# Autodesk Inventor assembly: Bed
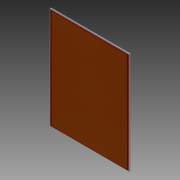
[picture p0: Inventor's stored thumbnail of the model, 180x180]
Saved by Autodesk Inventor 2015 (Build 190159000, 159)
## iProperties
Created: 2014-08-02
Part Number: Bed
Document SubType Name: Assembly
Designer: Jack
Author: Jack
## Documents named in this file (4)
- C:\Users\Jack\ownCloud\Projects\Core{XY}\InventorModel\Hardware\Bed\Bed.iam
- C:\Users\Jack\ownCloud\Projects\Core{XY}\InventorModel\Hardware\Bed\BedGlass.ipt
- C:\Users\Jack\ownCloud\Projects\Core{XY}\InventorModel\Hardware\Bed\HeatSpreader.ipt
- C:\Users\Jack\ownCloud\Projects\Core{XY}\InventorModel\Hardware\Bed\KaptonHeater.ipt
## Components (3 placed, 3 different names)
1. BedGlass:1 — Mate:1, Flush:3, Flush:4
2. HeatSpreader:1 — Mate:1, Mate:2, Flush:1, Flush:2, Flush:3, Flush:4
3. KaptonHeater:1 — Mate:2, Mate:3, Mate:4, Mate:5, Flush:1, Flush:2
## Relationships (9: Mate 5, Flush 4)
- Mate:1: BedGlass:1 ↔ HeatSpreader:1
- Mate:2: HeatSpreader:1 ↔ KaptonHeater:1
- Mate:3: KaptonHeater:1
- Mate:4: KaptonHeater:1
- Mate:5: KaptonHeater:1
- Flush:1 (2 mm): HeatSpreader:1 ↔ KaptonHeater:1
- Flush:2 (-4.5 mm): HeatSpreader:1 ↔ KaptonHeater:1
- Flush:3 (-3 mm): BedGlass:1 ↔ HeatSpreader:1
- Flush:4 (-3 mm): BedGlass:1 ↔ HeatSpreader:1
